# Autodesk Inventor assembly: grapplinghook
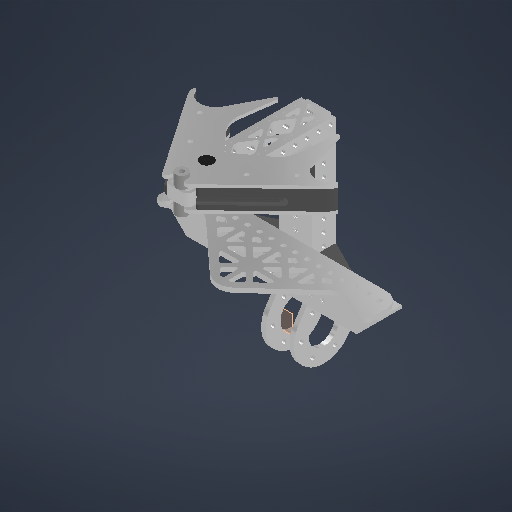
[picture p0: Inventor's stored thumbnail of the model, 512x512]
Saved by Autodesk Inventor 2025.1 (Build 291241020, 241B)
## iProperties
Category: _
Manager: _
ILogicPurgeVersion: 0.0.0.0
OnSaveVersion: 3.2.6.0
OnSaveAssembly: COREAutomationManager
Created: 2025-03-18
Part Number: grapplinghook
Checked By: 00
Engr Approved By: _
User Status: Work In Process
Description: ASSY,STANDARD (mm)
Document SubType Name: Assembly
Mfg Approved By: Paul.Struhar
Designer: mathe
Mass: 750.551 g
Surface Area: 2213.76 cm^2
Volume: 342.304 cm^3
Density: 2.19265 g/cm^3
CN_MASS: 0
CN_SERVICEABLE: _
FIRST_DESCRIPTION: _
SECOND_DESCRIPTION: _
THIRD_DESCRIPTION: _
CL_runCount: 0
ModelCat: Uncategorized
Subject: _
Author: mathe
Keywords: -
Revision Number: A
## Documents named in this file (13)
- D:\Documents\Inventor\2025-Poseidon-Mechanical\grapplinghook.iam
- D:\Documents\Inventor\2025-Poseidon-Mechanical\climber-arm-brace.ipt
- D:\Documents\Inventor\2025-Poseidon-Mechanical\climber-main-arm.ipt
- D:\Documents\Inventor\2025-Poseidon-Mechanical\climber-arm-middle-bar.ipt
- D:\Documents\Inventor\2025-Poseidon-Mechanical\grapple-pivot-shaft.ipt
- D:\Documents\Inventor\2025-Poseidon-Mechanical\grapple-spacer-thin.ipt
- D:\Documents\Inventor\2025-Poseidon-Mechanical\hook-top-plate.ipt
- D:\Documents\Inventor\2025-Poseidon-Mechanical\climber-hook-block.ipt
- D:\Documents\Inventor\2025-Poseidon-Mechanical\hook-bottom-plate.ipt
- D:\Documents\Inventor\2025-Poseidon-Mechanical\grapple-spacer-hardstop.ipt
- D:\Documents\Inventor\2025-Poseidon-Mechanical\cage-brace-support-bracket.ipt
- D:\Documents\Inventor\2025-Poseidon-Mechanical\cage-brace-arm.ipt
- D:\Documents\Inventor\2025-Poseidon-Mechanical\cage-brace.ipt
## Components (20 placed, 12 different names)
1. climber-arm-brace:1 — Mate:1, Flush:1, Flush:3, Mate:2, Flush:4, Flush:5, Flush:6, Flush:8, Insert:19, Flush:9
2. climber-main-arm:1 — Mate:2, Flush:4, Flush:5, Mate:3, Flush:7, Insert:20
3. climber-arm-brace:2 — Mate:3, Flush:6, Flush:7, Insert:1, Insert:18, Flush:10
4. climber-arm-middle-bar:1 — Insert:1, Flush:8, Insert:2, Insert:3, Insert:4, Insert:16, Insert:17
5. grapple-pivot-shaft:1 — Insert:2
6. grapple-spacer-thin:1 — Insert:3
7. hook-top-plate:1 — Insert:4, Insert:5, Insert:7, Insert:8
8. grapple-spacer-thin:2 — Insert:5, Insert:6
9. hook-top-plate:2 — Insert:6, Insert:9, Insert:10
10. climber-hook-block:1 — Insert:7, Insert:8, Insert:13, Insert:14
11. climber-hook-block:2 — Insert:9, Insert:10, Insert:11, Insert:12
12. hook-bottom-plate:1 — Insert:11, Insert:12, Insert:15
13. hook-bottom-plate:2 — Insert:13, Insert:14
14. grapple-spacer-thin:3 — Insert:15
15. grapple-spacer-hardstop:1 — Insert:16
16. grapple-spacer-hardstop:2 — Insert:17
17. cage-brace-support-bracket:1 — Insert:18, Flush:10
18. cage-brace-support-bracket:2 — Insert:19, Flush:9, Insert:21
19. cage-brace-arm:1 — Insert:20, Insert:21, Mate:4, Flush:11, Flush:12
20. cage-brace:1 — Mate:4, Flush:11, Flush:12
## Relationships (37: Insert 21, Flush 12, Mate 4)
- Mate:1: climber-arm-brace:1
- Flush:1: climber-arm-brace:1
- Flush:2 (12.7 mm)
- Flush:3: climber-arm-brace:1
- Mate:2: climber-arm-brace:1 ↔ climber-main-arm:1
- Flush:4 (12.7 mm): climber-arm-brace:1 ↔ climber-main-arm:1
- Flush:5: climber-arm-brace:1 ↔ climber-main-arm:1
- Mate:3: climber-main-arm:1 ↔ climber-arm-brace:2
- Flush:6: climber-arm-brace:1 ↔ climber-arm-brace:2
- Flush:7: climber-main-arm:1 ↔ climber-arm-brace:2
- Insert:1: climber-arm-brace:2 ↔ climber-arm-middle-bar:1
- Flush:8: climber-arm-brace:1 ↔ climber-arm-middle-bar:1
- Insert:2 (-11.1125 mm): climber-arm-middle-bar:1 ↔ grapple-pivot-shaft:1
- Insert:3: climber-arm-middle-bar:1 ↔ grapple-spacer-thin:1
- Insert:4: climber-arm-middle-bar:1 ↔ hook-top-plate:1
- Insert:5: hook-top-plate:1 ↔ grapple-spacer-thin:2
- Insert:6: grapple-spacer-thin:2 ↔ hook-top-plate:2
- Insert:7: hook-top-plate:1 ↔ climber-hook-block:1
- Insert:8: hook-top-plate:1 ↔ climber-hook-block:1
- Insert:9: hook-top-plate:2 ↔ climber-hook-block:2
- Insert:10: hook-top-plate:2 ↔ climber-hook-block:2
- Insert:11: climber-hook-block:2 ↔ hook-bottom-plate:1
- Insert:12: climber-hook-block:2 ↔ hook-bottom-plate:1
- Insert:13: climber-hook-block:1 ↔ hook-bottom-plate:2
- Insert:14: climber-hook-block:1 ↔ hook-bottom-plate:2
- Insert:15: hook-bottom-plate:1 ↔ grapple-spacer-thin:3
- Insert:16: climber-arm-middle-bar:1 ↔ grapple-spacer-hardstop:1
- Insert:17: climber-arm-middle-bar:1 ↔ grapple-spacer-hardstop:2
- Insert:18: climber-arm-brace:2 ↔ cage-brace-support-bracket:1
- Insert:19: climber-arm-brace:1 ↔ cage-brace-support-bracket:2
- Flush:9: climber-arm-brace:1 ↔ cage-brace-support-bracket:2
- Flush:10: climber-arm-brace:2 ↔ cage-brace-support-bracket:1
- Insert:20: climber-main-arm:1 ↔ cage-brace-arm:1
- Insert:21: cage-brace-support-bracket:2 ↔ cage-brace-arm:1
- Mate:4: cage-brace-arm:1 ↔ cage-brace:1
- Flush:11: cage-brace-arm:1 ↔ cage-brace:1
- Flush:12: cage-brace-arm:1 ↔ cage-brace:1
